# Autodesk Inventor assembly: EL2-C-300
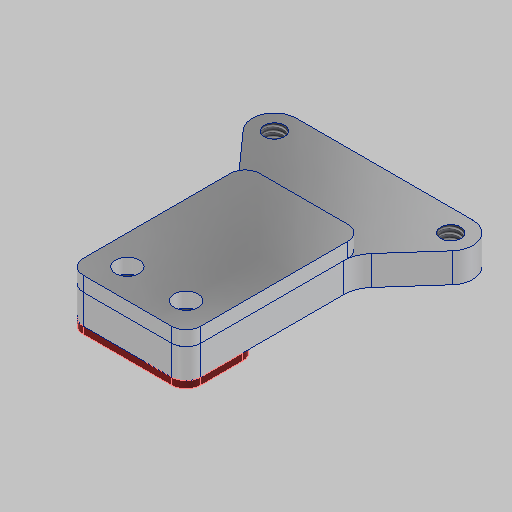
[picture p0: Inventor's stored thumbnail of the model, 512x512]
Saved by Autodesk Inventor 2023.5 (Build 275446000, 446)
## iProperties
Created: 2025-02-15
Part Number: EL2-C-300
Document SubType Name: Assembly
Designer: slick
Author: slick
## Documents named in this file (4)
- C:\Users\slick\OneDrive\Desktop\2025-ReefScape---CAD\Elevator\EL2\EL2-C-300.iam
- C:\Users\slick\OneDrive\Desktop\2025-ReefScape---CAD\Elevator\EL2\EL2-033.ipt
- C:\Users\slick\OneDrive\Desktop\2025-ReefScape---CAD\Elevator\EL2\EL2-019.ipt
- C:\Users\slick\OneDrive\Desktop\2025-ReefScape---CAD\Elevator\EL2\EL2-035.ipt
## Components (3 placed, 3 different names)
1. EL2-033:1 — Insert:1, Insert:2
2. EL2-019:1 — Insert:1, Insert:2, Insert:3, Insert:4
3. EL2-035:1 — Insert:3, Insert:4
## Relationships (4: Insert 4)
- Insert:1: EL2-033:1 ↔ EL2-019:1
- Insert:2: EL2-033:1 ↔ EL2-019:1
- Insert:3: EL2-019:1 ↔ EL2-035:1
- Insert:4: EL2-019:1 ↔ EL2-035:1
